# Autodesk Inventor assembly: Camera
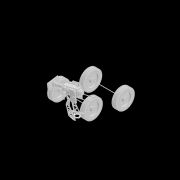
[picture p0: Inventor's stored thumbnail of the model, 180x180]
Saved by Autodesk Inventor 2020.4 (Build 244396010, 396A)
## iProperties
Created: 2022-09-19
Part Number: Camera
Document SubType Name: Assembly
Designer: Val
Author: Val
## Documents named in this file (10)
- C:\Users\Val\Desktop\tau\quote\Camera.iam
- C:\Users\Val\Desktop\tau\quote\Body.ipt
- C:\Users\Val\Desktop\tau\quote\BodyMirror.ipt
- C:\Users\Val\Desktop\tau\quote\S1.ipt
- C:\Users\Val\Desktop\tau\quote\S2.ipt
- C:\Users\Val\Desktop\tau\quote\CameraBody.ipt
- C:\Users\Val\Downloads\2481T51_Rubber Solid-Tread Flat-Free Wheel on Aluminum Core.ipt
- C:\Users\Val\Desktop\tau\external\TopHandle.ipt
- C:\Users\Val\Desktop\tau\MuzzleTube.ipt
- C:\Users\Val\Desktop\drummingrobot\src\parts\TorsoMount.ipt
## Components (15 placed, 9 different names)
1. Body:1 — Flush:2, Flush:3, Mate:11, Mate:32, Flush:11
2. BodyMirror:1 — Flush:2, Flush:3, Mate:12, Mate:33
3. S1:1 — Mate:13, Flush:4, Mate:15, Angle:3
4. S2:1 — Mate:14, Flush:4, Mate:15, Mate:34
5. CameraBody:1 — Mate:11, Mate:12, Mate:13, Mate:14, Mate:17, Angle:1, Angle:3, Flush:11
6. 2481T51_Rubber Solid-Tread Flat-Free Wheel on Aluminum Core:1 — Mate:29, Flush:6, Flush:12
7. 2481T51_Rubber Solid-Tread Flat-Free Wheel on Aluminum Core:2 — Mate:28, Flush:7
8. 2481T51_Rubber Solid-Tread Flat-Free Wheel on Aluminum Core:3 — Mate:30, Flush:9, Flush:12
9. 2481T51_Rubber Solid-Tread Flat-Free Wheel on Aluminum Core:4 — Mate:31, Flush:8
10. TopHandle:1 — Mate:17, Angle:1
11. MuzzleTube:4 — Mate:28, Mate:29, Flush:6, Flush:7
12. MuzzleTube:5 — Mate:30, Mate:31, Flush:8, Flush:9
13. MuzzleTube:6 — Mate:32, Flush:10
14. MuzzleTube:7 — Mate:33, Flush:10
15. TorsoMount:1 — Mate:34
## Relationships (25: Mate 13, Flush 10, Angle 2)
- Flush:2: Body:1 ↔ BodyMirror:1
- Flush:3: Body:1 ↔ BodyMirror:1
- Mate:11: Body:1 ↔ CameraBody:1
- Mate:12: BodyMirror:1 ↔ CameraBody:1
- Mate:13: S1:1 ↔ CameraBody:1
- Mate:14: S2:1 ↔ CameraBody:1
- Flush:4: S1:1 ↔ S2:1
- Mate:15: S1:1 ↔ S2:1
- Mate:17: CameraBody:1 ↔ TopHandle:1
- Angle:1 (0 deg): CameraBody:1 ↔ TopHandle:1
- Mate:28: 2481T51_Rubber Solid-Tread Flat-Free Wheel on Aluminum Core:2 ↔ MuzzleTube:4
- Mate:29: 2481T51_Rubber Solid-Tread Flat-Free Wheel on Aluminum Core:1 ↔ MuzzleTube:4
- Flush:6: 2481T51_Rubber Solid-Tread Flat-Free Wheel on Aluminum Core:1 ↔ MuzzleTube:4
- Flush:7: 2481T51_Rubber Solid-Tread Flat-Free Wheel on Aluminum Core:2 ↔ MuzzleTube:4
- Mate:30: 2481T51_Rubber Solid-Tread Flat-Free Wheel on Aluminum Core:3 ↔ MuzzleTube:5
- Mate:31: 2481T51_Rubber Solid-Tread Flat-Free Wheel on Aluminum Core:4 ↔ MuzzleTube:5
- Flush:8: 2481T51_Rubber Solid-Tread Flat-Free Wheel on Aluminum Core:4 ↔ MuzzleTube:5
- Flush:9: 2481T51_Rubber Solid-Tread Flat-Free Wheel on Aluminum Core:3 ↔ MuzzleTube:5
- Mate:32: Body:1 ↔ MuzzleTube:6
- Mate:33: BodyMirror:1 ↔ MuzzleTube:7
- Mate:34: S2:1 ↔ TorsoMount:1
- Flush:10: MuzzleTube:6 ↔ MuzzleTube:7
- Angle:3 (0 deg): S1:1 ↔ CameraBody:1
- Flush:11: Body:1 ↔ CameraBody:1
- Flush:12: 2481T51_Rubber Solid-Tread Flat-Free Wheel on Aluminum Core:1 ↔ 2481T51_Rubber Solid-Tread Flat-Free Wheel on Aluminum Core:3
